# Autodesk Inventor assembly: ArmAssembly
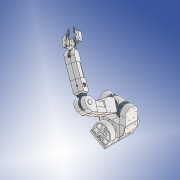
[picture p0: Inventor's stored thumbnail of the model, 180x180]
Saved by Autodesk Inventor 2017 (Build 210142000, 142)
## iProperties
Created: 2017-05-10
Part Number: ArmAssembly
Document SubType Name: Assembly
Designer: zallen
Author: zallen
## Documents named in this file (5)
- C:\Users\zallen\Documents\GitHub\cr-laundry-robot\src\Body 2\Arm Assembly\ArmAssembly.iam
- C:\Users\zallen\Documents\GitHub\cr-laundry-robot\src\Body 2\Arm Assembly\Shoulder Joint Assembly\Shoulder Joint Assembly.iam
- C:\Users\zallen\Documents\GitHub\cr-laundry-robot\src\Body 2\Arm Assembly\Bicep Assembly\BicepAssembly.iam
- C:\Users\zallen\Documents\GitHub\cr-laundry-robot\src\Body 2\Arm Assembly\Fore Arm Assembly\ForeArmAssembly.iam
- C:\Users\zallen\Documents\GitHub\cr-laundry-robot\src\Body 2\Arm Assembly\Gripper Assembly\Gripper Assembly.iam
## Components (4 placed, 4 different names)
1. Shoulder Joint Assembly:1 [sub-assembly] — Mate:67, Mate:68, Mate:69, Mate:78, Mate:79
2. BicepAssembly:1 [sub-assembly] — Mate:72, Mate:73, Mate:78, Mate:79
3. ForeArmAssembly:1 [sub-assembly] — Mate:72, Mate:73, Mate:75, Mate:76
4. Gripper Assembly:1 [sub-assembly] — Mate:75, Mate:76
## Relationships (9: Mate 9)
- Mate:67: Shoulder Joint Assembly:1
- Mate:68: Shoulder Joint Assembly:1
- Mate:69: Shoulder Joint Assembly:1
- Mate:72: BicepAssembly:1 ↔ ForeArmAssembly:1
- Mate:73: BicepAssembly:1 ↔ ForeArmAssembly:1
- Mate:75: ForeArmAssembly:1 ↔ Gripper Assembly:1
- Mate:76: ForeArmAssembly:1 ↔ Gripper Assembly:1
- Mate:78: Shoulder Joint Assembly:1 ↔ BicepAssembly:1
- Mate:79: Shoulder Joint Assembly:1 ↔ BicepAssembly:1
